# Autodesk Inventor assembly: SS cylinder block
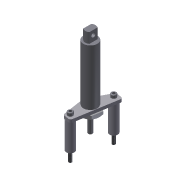
[picture p0: Inventor's stored thumbnail of the model, 180x180]
Saved by Autodesk Inventor 2011 (Build 150239000, 239)
## iProperties
Created: 2011-07-04
Part Number: SS cylinder block
Document SubType Name: Assembly
Designer: Dan Niemitalo
Translation Standard: STEP AP203
FileName: //Amserv/amserver/AndyMark/Products/Gearboxes Shifters/Super Shifter/super-shifter-asm-penumatic-motor-cyl.stp
PreProcessor: Unknown
PostProcessor: Build: 282, Release: 2011 SP1 - Date: Thu 08/05/2010
Sent Units: millimeter
Uncertainty: 0.001
Author: Dan Niemitalo
## Documents named in this file (7)
- H:\Nemo\Documents\Robotics\COTS Parts\Gearboxes\Shifters\Shifter Cylinder Subassembly.iam
- H:\Nemo\Documents\Robotics\COTS Parts\Fasteners\58-18 jam nut.ipt
- H:\Nemo\Documents\Robotics\COTS Parts\Gearboxes\Shifters\Shifter cylinder block spacer.ipt
- H:\Nemo\Documents\Robotics\COTS Parts\Gearboxes\Shifters\Cylinder for shifters.ipt
- H:\Nemo\Documents\Robotics\COTS Parts\Gearboxes\Shifters\Shifter cylinder plate.ipt
- H:\Nemo\Documents\Robotics\COTS Parts\Fasteners\14-28 jam nut.ipt
- H:\Nemo\Documents\Robotics\COTS Parts\Fasteners\10-32 SHCS x2500.ipt
## Components (8 placed, 6 different names)
1. Shifter cylinder block spacer:1 — Insert:4
2. Shifter cylinder block spacer:2 — Insert:3
3. Shifter cylinder plate:1 — Insert:1, Insert:2, Insert:3, Insert:4, Insert:5, Insert:6
4. 14-28 jam nut:1 — Insert:7
5. 58-18 jam nut:1 — Insert:2
6. Cylinder for shifters:1 — Mate:1, Mate:2, Angle:1, Insert:1, Insert:7
7. 10-32 SHCS x2500:1 — Insert:6
8. 10-32 SHCS x2500:2 — Insert:5
## Relationships (10: Insert 7, Mate 2, Angle 1)
- Mate:1: Cylinder for shifters:1
- Mate:2: Cylinder for shifters:1
- Angle:1 (0 deg): Cylinder for shifters:1
- Insert:1: Shifter cylinder plate:1 ↔ Cylinder for shifters:1
- Insert:2: Shifter cylinder plate:1 ↔ 58-18 jam nut:1
- Insert:3: Shifter cylinder block spacer:2 ↔ Shifter cylinder plate:1
- Insert:4: Shifter cylinder block spacer:1 ↔ Shifter cylinder plate:1
- Insert:5: Shifter cylinder plate:1 ↔ 10-32 SHCS x2500:2
- Insert:6: Shifter cylinder plate:1 ↔ 10-32 SHCS x2500:1
- Insert:7: 14-28 jam nut:1 ↔ Cylinder for shifters:1
